# Autodesk Inventor assembly: Extruder Mechanism
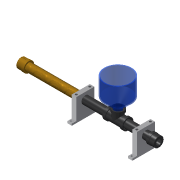
[picture p0: Inventor's stored thumbnail of the model, 180x180]
Saved by Autodesk Inventor 2014 SP1 (Build 180222100, 222)
## iProperties
Created: 2014-12-05
Part Number: Extruder Mechanism
Document SubType Name: Assembly
Designer: AlecShufelt
Mass: 337.565 g
Surface Area: 1255.02 cm^2
Volume: 217.444 cm^3
Density: 1.55242 g/cm^3
Author: AlecShufelt
## Documents named in this file (9)
- C:\Users\AlecShufelt\Documents\Drafting\CEMS Research\Prototype 2.0\Extruder Mechanism.iam
- C:\Users\AlecShufelt\Documents\Drafting\CEMS Research\Prototype 2.0\Pipe.ipt
- C:\Users\AlecShufelt\Documents\Drafting\CEMS Research\Prototype 2.0\Pipe T.ipt
- C:\Users\AlecShufelt\Documents\Drafting\CEMS Research\Prototype 2.0\Pipe Cap.ipt
- C:\Users\AlecShufelt\Documents\Drafting\CEMS Research\Prototype 2.0\Pipe bracket.ipt
- C:\Users\AlecShufelt\Documents\Drafting\CEMS Research\Prototype 2.0\Pipe2.ipt
- C:\Users\AlecShufelt\Documents\Drafting\CEMS Research\Prototype 2.0\Thermal Tape.ipt
- C:\Users\AlecShufelt\Documents\Drafting\CEMS Research\Prototype 2.0\Hopper.ipt
- C:\Users\AlecShufelt\Documents\Drafting\CEMS Research\Prototype 2.0\Pipe Cap 3 - Kapton Tape.ipt
## Components (9 placed, 8 different names)
1. Pipe:1 — Insert:1, Insert:9, Insert:14, Insert:16
2. Pipe T:1 — Insert:1, Insert:8, Insert:9, Insert:13
3. Pipe2:1 — Insert:7, Insert:8, Insert:15
4. Pipe Cap:2 — Insert:7
5. Thermal Tape:1 — Insert:16, Insert:17
6. Hopper:1 — Insert:13
7. Pipe bracket:1 — Insert:14
8. Pipe bracket:2 — Insert:15
9. Pipe Cap 3 - Kapton Tape:1 — Insert:17
## Relationships (9: Insert 9)
- Insert:1: Pipe:1 ↔ Pipe T:1
- Insert:7: Pipe2:1 ↔ Pipe Cap:2
- Insert:8: Pipe T:1 ↔ Pipe2:1
- Insert:9: Pipe:1 ↔ Pipe T:1
- Insert:13: Pipe T:1 ↔ Hopper:1
- Insert:14 (-76.2 mm): Pipe:1 ↔ Pipe bracket:1
- Insert:15 (-50.8 mm): Pipe2:1 ↔ Pipe bracket:2
- Insert:16: Pipe:1 ↔ Thermal Tape:1
- Insert:17: Thermal Tape:1 ↔ Pipe Cap 3 - Kapton Tape:1
